# Autodesk Inventor assembly: gear
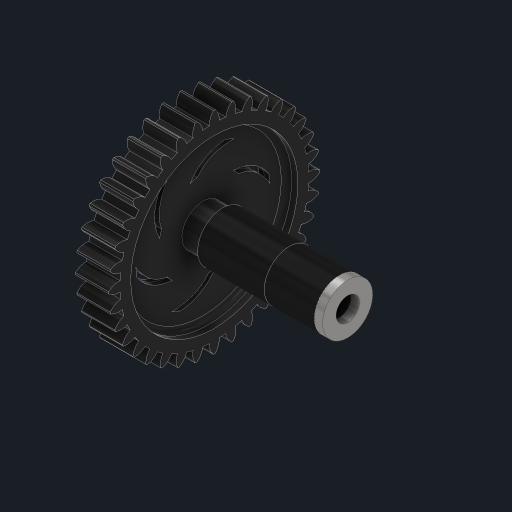
[picture p0: Inventor's stored thumbnail of the model, 512x512]
Saved by Autodesk Inventor 2024 (Build 280153000, 153)
## iProperties
Created: 2024-03-23
Part Number: gear
Document SubType Name: Assembly
Designer: Averey Ku
Author: Averey Ku
## Documents named in this file (7)
- D:\vex_robotics\hardware\cad\infection\chassis\drivebay\gear.iam
- D:\vex_robotics\hardware\cad\VEX-CAD-Inventor-1.41\Motion\Gears\LS 36T Gear.ipt
- D:\vex_robotics\hardware\cad\VEX-CAD-Inventor-1.41\Motion\Spacers\Spacer Nylon .375 OD.ipt
- D:\vex_robotics\hardware\cad\VEX-CAD-Inventor-1.41\Motion\Spacers\Spacer Nylon .375 OD\NSpacer .375 OD x .375.ipt
- D:\vex_robotics\hardware\cad\VEX-CAD-Inventor-1.41\Motion\Spacers\Spacer Nylon .375 OD\NSpacer .375 OD x .500.ipt
- D:\vex_robotics\hardware\cad\VEX-CAD-Inventor-1.41\Motion\Spacers\Washer Steel\SWasher .375 OD x .062500.ipt
- D:\vex_robotics\hardware\cad\VEX-CAD-Inventor-1.41\Motion\Spacers\Washer Steel.ipt
## Components (5 placed, 4 different names)
1. LS 36T Gear:1 — Insert:2, Insert:4
2. NSpacer .375 OD x .375:2 — Insert:1, Insert:3
3. NSpacer .375 OD x .500:3 — Insert:1, Insert:4
4. SWasher .375 OD x .062500:1 — Insert:3
5. SWasher .375 OD x .062500:2 — Insert:2
## Relationships (4: Insert 4)
- Insert:1: NSpacer .375 OD x .375:2 ↔ NSpacer .375 OD x .500:3
- Insert:2: LS 36T Gear:1 ↔ SWasher .375 OD x .062500:2
- Insert:3: NSpacer .375 OD x .375:2 ↔ SWasher .375 OD x .062500:1
- Insert:4: LS 36T Gear:1 ↔ NSpacer .375 OD x .500:3
